# Autodesk Inventor assembly: gear_motor
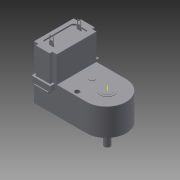
[picture p0: Inventor's stored thumbnail of the model, 180x180]
Saved by Autodesk Inventor 2014 (Build 180170000, 170)
## iProperties
Created: 2013-06-25
Part Number: gear_motor
Document SubType Name: Assembly
Designer: Felix
Author: Felix
## Documents named in this file (5)
- C:\Users\Felix\Desktop\Pololu_gear_motor_1_180\gear_motor.iam
- C:\Users\Felix\Desktop\Pololu_gear_motor_1_180\front.ipt
- C:\Users\Felix\Desktop\Pololu_gear_motor_1_180\motor_shaft.ipt
- C:\Users\Felix\Desktop\Pololu_gear_motor_1_180\wheel_shaft.ipt
- C:\Users\Felix\Desktop\Pololu_gear_motor_1_180\motor_contact.ipt
## Components (5 placed, 4 different names)
1. front:1 — Passend:1, Fluchtend:1, Fluchtend:2, Passend:2, Passend:3, Passend:8, Passend:9, Passend:10
2. motor_shaft:1 — Passend:1, Fluchtend:1, Fluchtend:2, Passend:4, Passend:5, Passend:6, Passend:7, Fluchtend:3, Fluchtend:4
3. wheel_shaft:1 — Passend:2, Passend:3
4. motor_contact:1 — Passend:5, Passend:7, Fluchtend:3
5. motor_contact:2 — Passend:4, Passend:6, Fluchtend:4
## Relationships (14: Mate 10, Flush 4)
- Passend:1 [Mate]: front:1 ↔ motor_shaft:1
- Fluchtend:1 [Flush]: front:1 ↔ motor_shaft:1
- Fluchtend:2 [Flush]: front:1 ↔ motor_shaft:1
- Passend:2 [Mate]: front:1 ↔ wheel_shaft:1
- Passend:3 [Mate]: front:1 ↔ wheel_shaft:1
- Passend:4 [Mate]: motor_shaft:1 ↔ motor_contact:2
- Passend:5 [Mate]: motor_shaft:1 ↔ motor_contact:1
- Passend:6 [Mate] (-4.5 mm): motor_shaft:1 ↔ motor_contact:2
- Passend:7 [Mate] (-4.5 mm): motor_shaft:1 ↔ motor_contact:1
- Fluchtend:3 [Flush] (-4.5 mm): motor_shaft:1 ↔ motor_contact:1
- Fluchtend:4 [Flush] (-4.5 mm): motor_shaft:1 ↔ motor_contact:2
- Passend:8 [Mate]: front:1
- Passend:9 [Mate]: front:1
- Passend:10 [Mate]: front:1
